# Autodesk Inventor assembly: Body
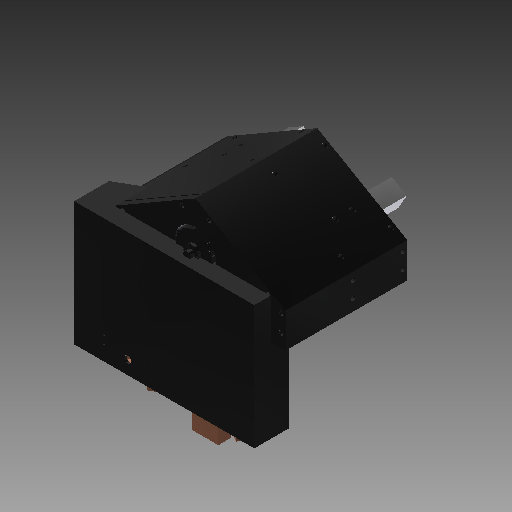
[picture p0: Inventor's stored thumbnail of the model, 512x512]
Saved by Autodesk Inventor 2017 (Build 210142000, 142)
## iProperties
Created: 2018-10-18
Part Number: Body
Document SubType Name: Assembly
Designer: Dell
Author: Dell
## Documents named in this file (6)
- C:\Users\Dell\Documents\GitHub\tr2\Body\Body.iam
- C:\Users\Dell\Documents\GitHub\tr2\Body\Body Cover Assembly.iam
- C:\Users\Dell\Documents\GitHub\tr2\Body\Body Chassis Assembly.iam
- C:\Users\Dell\Documents\GitHub\tr2\Body\BO13.ipt
- C:\Users\Dell\Documents\GitHub\tr2\Actuator 1.2\Actuator 1.2.iam
- C:\Users\Dell\Documents\GitHub\tr2\Body\HDPE Body.iam
## Components (5 placed, 5 different names)
1. Body Cover Assembly:1 [sub-assembly] — Mate:72, Mate:78, Mate:92
2. Body Chassis Assembly:1 [sub-assembly] — Mate:72, Mate:78, Mate:79, Mate:85, Mate:86, Mate:87, Flush:2, Flush:3, Mate:91, Mate:92
3. BO13:1 — Mate:79, Mate:88, Mate:89, Flush:3, Mate:90, Mate:91
4. Actuator 1.2:1 [sub-assembly] — Mate:88, Mate:89, Mate:90
5. HDPE Body:1 [sub-assembly]
## Relationships (13: Mate 11, Flush 2)
- Mate:72: Body Cover Assembly:1 ↔ Body Chassis Assembly:1
- Mate:78: Body Cover Assembly:1 ↔ Body Chassis Assembly:1
- Mate:79: Body Chassis Assembly:1 ↔ BO13:1
- Mate:85: Body Chassis Assembly:1
- Mate:86: Body Chassis Assembly:1
- Mate:87: Body Chassis Assembly:1
- Flush:2: Body Chassis Assembly:1
- Mate:88: BO13:1 ↔ Actuator 1.2:1
- Mate:89: BO13:1 ↔ Actuator 1.2:1
- Flush:3 (-182 mm): Body Chassis Assembly:1 ↔ BO13:1
- Mate:90: BO13:1 ↔ Actuator 1.2:1
- Mate:91: Body Chassis Assembly:1 ↔ BO13:1
- Mate:92: Body Cover Assembly:1 ↔ Body Chassis Assembly:1
